# Autodesk Inventor assembly: fab model mk-1
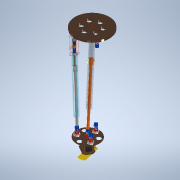
[picture p0: Inventor's stored thumbnail of the model, 180x180]
Saved by Autodesk Inventor 2020 (Build 240168000, 168)
## iProperties
Created: 2020-12-19
Part Number: fab model mk-1
Document SubType Name: Assembly
Designer: Vikki
Author: Vikki
## Documents named in this file (24)
- E:\borewell rescuebot\pll manipulator files\sps manipulator\fab model mk-2.iam
- E:\borewell rescuebot\pll manipulator files\sps manipulator\base.ipt
- E:\borewell rescuebot\pll manipulator files\sps manipulator\craftsman-3-pc-universal-joint-set-1.snapshot.1\Craftsman Socket U-Joint.iam
- E:\borewell rescuebot\pll manipulator files\sps manipulator\platform.ipt
- E:\borewell rescuebot\pll manipulator files\sps manipulator\leadscrew.ipt
- E:\borewell rescuebot\pll manipulator files\sps manipulator\coupler.ipt
- E:\borewell rescuebot\pll manipulator files\sps manipulator\telescopic boom1.ipt
- E:\borewell rescuebot\pll manipulator files\sps manipulator\boom 3.ipt
- E:\borewell rescuebot\pll manipulator files\sps manipulator\ball-pin.ipt
- E:\borewell rescuebot\2020 bot\borewell max sixe.ipt
- E:\borewell rescuebot\2020 bot\min size bore well.ipt
- E:\borewell rescuebot\pll manipulator files\sps manipulator\fab model mk-1\Design Accelerator\Bearing1.iam
- E:\borewell rescuebot\pll manipulator files\sps manipulator\MicroGearmotor v3.ipt
- E:\borewell rescuebot\pll manipulator files\sps manipulator\plunger.ipt
- E:\borewell rescuebot\pll manipulator files\sps manipulator\piston.ipt
- E:\borewell rescuebot\pll manipulator files\sps manipulator\fab model mk-2\Design Accelerator\Bearing1.iam
- E:\borewell rescuebot\pll manipulator files\sps manipulator\fab model mk-2\Design Accelerator\Bearing2.iam
- E:\borewell rescuebot\pll manipulator files\sps manipulator\motor bracket n 20.ipt
- E:\borewell rescuebot\pll manipulator files\sps manipulator\female joint for uv.ipt
- E:\borewell rescuebot\pll manipulator files\sps manipulator\platform uv femal joint.ipt
- E:\borewell rescuebot\pll manipulator files\sps manipulator\boom to female.ipt
- E:\borewell rescuebot\pll manipulator files\sps manipulator\servo mg958 dummy.ipt
- E:\borewell rescuebot\pll manipulator files\sps manipulator\z roto base.ipt
- E:\borewell rescuebot\pll manipulator files\sps manipulator\MG-958 servo.iam
## Components (37 placed, 21 different names)
1. base:1 — Mate:1, Mate:2, Mate:3, Mate:4, Mate:5, Mate:6, Angle:1, Mate:18, Mate:19, Mate:61, Flush:6, M1 C, M2 C
2. Craftsman Socket U-Joint:1 [sub-assembly] — Mate:1, Mate:2, Angle:2, Mate:90
3. Craftsman Socket U-Joint:2 [sub-assembly] — Mate:5, Mate:6, Angle:3, Mate:92
4. Craftsman Socket U-Joint:3 [sub-assembly] — Mate:3, Mate:4, Angle:1, Angle:2, Angle:3, Mate:23, Mate:91, Mate:93, Angle:7, Mate:108, Mate:109
5. platform:1 — Mate:7, Mate:9, Mate:10, Mate:16, Mate:17, Mate:63, Flush:8, Mate:64, Mate:65, Flush:9, Flush:10, M1 C, M2 C, Angle:6, Mate:128, Mate:130, Angle:15
6. Craftsman Socket U-Joint:4 [sub-assembly] — Mate:7, Mate:90, Mate:133
7. Craftsman Socket U-Joint:5 [sub-assembly] — Mate:9, Mate:91, Mate:111, Mate:112, Mate:132
8. Craftsman Socket U-Joint:6 [sub-assembly] — Mate:10, Mate:23, Mate:92, Mate:131
9. Craftsman Socket U-Joint:7 [sub-assembly] — Mate:16, Mate:17, Mate:26, Flush:1, Mate:60, Angle:6, Mate:100, Mate:101
10. Craftsman Socket U-Joint:8 [sub-assembly] — Mate:18, Mate:19, Angle:5, Mate:26, Flush:1, Mate:48, Mate:59, Mate:114, Mate:115
11. leadscrew:1 — Mate:37, Mate:38, Mate:97, Mate:103
12. coupler:1 — Mate:37, Mate:38, Mate:95, Mate:105, Mate:118, Mate:119
13. leadscrew:2 — Mate:40
14. coupler:2 — Mate:40
15. leadscrew:3
16. coupler:3
17. telescopic boom1:1 — Mate:48, Mate:59, Angle:12
18. boom 3:1 — Mate:100, Mate:101, Angle:12
19. ball-pin:1 — Mate:60
20. borewell max sixe:1 — Mate:61, Mate:62, Flush:5
21. min size bore well:1 — Mate:62, Flush:5, Flush:6
22. Bearing:1 [sub-assembly] — Mate:63, Flush:8, Mate:131
23. Bearing:2 [sub-assembly] — Mate:64, Flush:10, Mate:133
24. Bearing:3 [sub-assembly] — Mate:65, Flush:9, Mate:132
25. MicroGearmotor v3:1 — Mate:93, Angle:7, Mate:95, Mate:98, Angle:9, Mate:120
26. plunger:1 — Mate:97, Angle:11, Mate:113
27. piston:1 — Mate:98, Angle:10, Angle:11, Mate:117
28. Bearing:4 [sub-assembly] — Mate:103, Flush:13, Mate:119
29. Bearing:5 [sub-assembly] — Mate:105, Flush:12
30. motor bracket n 20:1 — Angle:9, Mate:110, Flush:12, Angle:10, Mate:117, Flush:13, Mate:118, Mate:120
31. female joint for uv:1 — Mate:108, Mate:109, Mate:110
32. platform uv femal joint:1 — Mate:111, Mate:112, Mate:113
33. boom to female:1 — Mate:114, Mate:115
34. servo mg958 dummy:1
35. MicroGearmotor v3:2 — Mate:125, Mate:126, Angle:14
36. z roto base:1 — Mate:125, Mate:126, Angle:14, Mate:127, Mate:129
37. MG-958 servo:1 [sub-assembly] — Mate:127, Mate:128, Mate:129, Mate:130, Angle:15
## Relationships (85: Mate 62, Angle 12, Flush 11)
- Mate:1: base:1 ↔ Craftsman Socket U-Joint:1
- Mate:2: base:1 ↔ Craftsman Socket U-Joint:1
- Mate:3: base:1 ↔ Craftsman Socket U-Joint:3
- Mate:4: base:1 ↔ Craftsman Socket U-Joint:3
- Mate:5: base:1 ↔ Craftsman Socket U-Joint:2
- Mate:6: base:1 ↔ Craftsman Socket U-Joint:2
- Mate:7: platform:1 ↔ Craftsman Socket U-Joint:4
- Mate:9: platform:1 ↔ Craftsman Socket U-Joint:5
- Mate:10: platform:1 ↔ Craftsman Socket U-Joint:6
- Angle:1 (30 deg): base:1 ↔ Craftsman Socket U-Joint:3
- Angle:2 (60 deg): Craftsman Socket U-Joint:1 ↔ Craftsman Socket U-Joint:3
- Angle:3 (120 deg): Craftsman Socket U-Joint:2 ↔ Craftsman Socket U-Joint:3
- Mate:16: platform:1 ↔ Craftsman Socket U-Joint:7
- Mate:17: platform:1 ↔ Craftsman Socket U-Joint:7
- Mate:18: base:1 ↔ Craftsman Socket U-Joint:8
- Mate:19: base:1 ↔ Craftsman Socket U-Joint:8
- Angle:5 (0 deg): Craftsman Socket U-Joint:8
- Mate:23: Craftsman Socket U-Joint:3 ↔ Craftsman Socket U-Joint:6
- Mate:26: Craftsman Socket U-Joint:7 ↔ Craftsman Socket U-Joint:8
- Flush:1: Craftsman Socket U-Joint:7 ↔ Craftsman Socket U-Joint:8
- Mate:37: leadscrew:1 ↔ coupler:1
- Mate:38 (-10 mm): leadscrew:1 ↔ coupler:1
- [Mate]: leadscrew:2 ↔ coupler:2
- Mate:40 (-10 mm): leadscrew:2 ↔ coupler:2
- [Mate]: leadscrew:3 ↔ coupler:3
- [Mate] (-10 mm): leadscrew:3 ↔ coupler:3
- Mate:48: Craftsman Socket U-Joint:8 ↔ telescopic boom1:1
- Mate:59 (-5 mm): Craftsman Socket U-Joint:8 ↔ telescopic boom1:1
- Mate:60: Craftsman Socket U-Joint:7 ↔ ball-pin:1
- [Flush]: borewell max sixe:1 ↔ min size bore well:1
- [Flush]: borewell max sixe:1 ↔ min size bore well:1
- Mate:61: base:1 ↔ borewell max sixe:1
- Mate:62: borewell max sixe:1 ↔ min size bore well:1
- Flush:5: borewell max sixe:1 ↔ min size bore well:1
- Flush:6 (-400 mm): base:1 ↔ min size bore well:1
- Mate:63: platform:1 ↔ Bearing:1
- Flush:8: platform:1 ↔ Bearing:1
- Mate:64: platform:1 ↔ Bearing:2
- Mate:65: platform:1 ↔ Bearing:3
- Flush:9: platform:1 ↔ Bearing:3
- Flush:10: platform:1 ↔ Bearing:2
- M1 C [Flush] (400 mm): base:1 ↔ platform:1
- M2 C [Mate]: base:1 ↔ platform:1
- Mate:90: Craftsman Socket U-Joint:1 ↔ Craftsman Socket U-Joint:4
- Mate:91: Craftsman Socket U-Joint:3 ↔ Craftsman Socket U-Joint:5
- Mate:92: Craftsman Socket U-Joint:2 ↔ Craftsman Socket U-Joint:6
- Angle:6 (30 deg): platform:1 ↔ Craftsman Socket U-Joint:7
- Mate:93: Craftsman Socket U-Joint:3 ↔ MicroGearmotor v3:1
- Angle:7 (0 deg): Craftsman Socket U-Joint:3 ↔ MicroGearmotor v3:1
- Mate:95: coupler:1 ↔ MicroGearmotor v3:1
- Mate:97: leadscrew:1 ↔ plunger:1
- Mate:98: MicroGearmotor v3:1 ↔ piston:1
- Mate:100: Craftsman Socket U-Joint:7 ↔ boom 3:1
- Mate:101: Craftsman Socket U-Joint:7 ↔ boom 3:1
- Mate:103: leadscrew:1 ↔ Bearing:4
- Mate:105: coupler:1 ↔ Bearing:5
- Angle:9 (0 deg): MicroGearmotor v3:1 ↔ motor bracket n 20:1
- Mate:108: Craftsman Socket U-Joint:3 ↔ female joint for uv:1
- Mate:109: Craftsman Socket U-Joint:3 ↔ female joint for uv:1
- Mate:110: motor bracket n 20:1 ↔ female joint for uv:1
- Flush:12: Bearing:5 ↔ motor bracket n 20:1
- Angle:10 (0 deg): piston:1 ↔ motor bracket n 20:1
- Angle:11 (0 deg): plunger:1 ↔ piston:1
- Mate:111: Craftsman Socket U-Joint:5 ↔ platform uv femal joint:1
- Mate:112: Craftsman Socket U-Joint:5 ↔ platform uv femal joint:1
- Mate:113: plunger:1 ↔ platform uv femal joint:1
- Angle:12 (0 deg): telescopic boom1:1 ↔ boom 3:1
- Mate:114: Craftsman Socket U-Joint:8 ↔ boom to female:1
- Mate:115: Craftsman Socket U-Joint:8 ↔ boom to female:1
- Mate:117: piston:1 ↔ motor bracket n 20:1
- Flush:13: Bearing:4 ↔ motor bracket n 20:1
- Mate:118: coupler:1 ↔ motor bracket n 20:1
- Mate:119: coupler:1 ↔ Bearing:4
- Mate:120: MicroGearmotor v3:1 ↔ motor bracket n 20:1
- Mate:125: MicroGearmotor v3:2 ↔ z roto base:1
- Mate:126: MicroGearmotor v3:2 ↔ z roto base:1
- Angle:14 (180 deg): MicroGearmotor v3:2 ↔ z roto base:1
- Mate:127: z roto base:1 ↔ MG-958 servo:1
- Mate:128: platform:1 ↔ MG-958 servo:1
- Mate:129 (3 mm): z roto base:1 ↔ MG-958 servo:1
- Mate:130: platform:1 ↔ MG-958 servo:1
- Angle:15 (0 deg): platform:1 ↔ MG-958 servo:1
- Mate:131: Craftsman Socket U-Joint:6 ↔ Bearing:1
- Mate:132: Craftsman Socket U-Joint:5 ↔ Bearing:3
- Mate:133: Craftsman Socket U-Joint:4 ↔ Bearing:2
## Named parameters: d70_d68 = 0 mm, d71_d69 = -10 mm, d72_d68 = 0 mm, d73_d69 = -10 mm
